# Autodesk Inventor assembly: accumulator and magnets
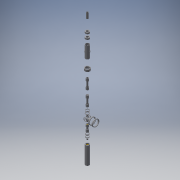
[picture p0: Inventor's stored thumbnail of the model, 180x180]
Saved by Autodesk Inventor 2019 (Build 230136000, 136)
## iProperties
Created: 2019-07-27
Part Number: accumulator and magnets
Document SubType Name: Assembly
Designer: afelepar
Author: afelepar
## Documents named in this file (4)
- G:\Experiments\ALPHA\Personal folders\Ali Fele Paranj\Inventor\Accumulator and magnets\files\accumulator and magnets.iam
- G:\Experiments\ALPHA\Personal folders\Ali Fele Paranj\Inventor\Accumulator and magnets\files\Acc_PenningTrap.iam
- G:\Experiments\ALPHA\Personal folders\Ali Fele Paranj\Inventor\Accumulator and magnets\files\magnets.iam
- G:\Experiments\ALPHA\Personal folders\Ali Fele Paranj\Inventor\Accumulator and magnets\files\buncher.iam
## Components (3 placed, 3 different names)
1. buncher:1 [sub-assembly] — Mate:4, Flush:2, Angle:1
2. Acc_PenningTrap:1 [sub-assembly] — Mate:1, Flush:1
3. magnets:1 [sub-assembly] — Mate:1, Flush:1, Mate:2, Mate:3, Flush:2
## Relationships (7: Mate 4, Flush 2, Angle 1)
- Mate:1: Acc_PenningTrap:1 ↔ magnets:1
- Flush:1: Acc_PenningTrap:1 ↔ magnets:1
- Mate:2: magnets:1
- Mate:3: magnets:1
- Mate:4: buncher:1
- Flush:2: buncher:1 ↔ magnets:1
- Angle:1 (180 deg): buncher:1
